# Autodesk Inventor assembly: ParticleLauncherwCollector
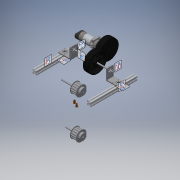
[picture p0: Inventor's stored thumbnail of the model, 180x180]
Saved by Autodesk Inventor 2016 (Build 200138000, 138)
## iProperties
Created: 2016-10-12
Part Number: ParticleLauncherwCollector
Document SubType Name: Assembly
Designer: Delta
Author: Delta
## Documents named in this file (11)
- C:\Robotics\CAD\2016-17_CAD\ParticleLauncherwCollector.iam
- C:\Robotics\CAD\COTSParts\Actobotics\555 parts\555116.ipt
- C:\Robotics\CAD\COTSParts\Actobotics\am-3102NeveRest20 (1).ipt
- C:\Robotics\CAD\COTSParts\Actobotics\634 parts\634088.ipt
- C:\Robotics\CAD\COTSParts\Wheels\4in Wheel Intergreated Hub 8mm Rev2.ipt
- C:\Robotics\CAD\COTSParts\Brecoflex\ls40t10_15-2_hub-32x10_d-8h7.ipt
- C:\Robotics\CAD\COTSParts\Actobotics\634 parts\634080.ipt
- C:\Robotics\CAD\COTSParts\Actobotics\634 parts\634078.ipt
- C:\Robotics\CAD\COTSParts\Bosch Extrusion\Bosch 20x20 9 in.ipt
- C:\Robotics\CAD\COTSParts\Actobotics\585 parts\585494.ipt
- C:\Robotics\CAD\COTSParts\Tetrix\Bronze bushing.ipt
## Components (15 placed, 10 different names)
1. 555116:1 — Insert:15
2. am-3102NeveRest20 (1):1 — Insert:15, Insert:18
3. 634088:1 — Insert:17, Insert:23, Insert:24
4. 4in Wheel Intergreated Hub 8mm Rev2:1 — Insert:17
5. 4in Wheel Intergreated Hub 8mm Rev2:2 — Insert:18
6. ls40t10_15-2_hub-32x10_d-8h7:1
7. ls40t10_15-2_hub-32x10_d-8h7:2
8. 634080:1
9. 634078:1
10. Bosch 20x20 9 in:1 — Mate:1, Flush:1, Flush:2
11. Bosch 20x20 9 in:2 — Mate:2, Flush:3
12. 585494:2 — Insert:23, Mate:1, Flush:1, Flush:2
13. 585494:3 — Insert:24, Mate:2, Flush:3
14. Bronze bushing:1
15. Bronze bushing:2
## Relationships (10: Insert 5, Flush 3, Mate 2)
- Insert:15 (-9.525 mm): 555116:1 ↔ am-3102NeveRest20 (1):1
- Insert:17 (76.2 mm): 634088:1 ↔ 4in Wheel Intergreated Hub 8mm Rev2:1
- Insert:18 (-19.05 mm): am-3102NeveRest20 (1):1 ↔ 4in Wheel Intergreated Hub 8mm Rev2:2
- Insert:23 (-12.7 mm): 634088:1 ↔ 585494:2
- Mate:1: Bosch 20x20 9 in:1 ↔ 585494:2
- Flush:1 (4.318 mm): Bosch 20x20 9 in:1 ↔ 585494:2
- Flush:2 (63.5 mm): Bosch 20x20 9 in:1 ↔ 585494:2
- Insert:24 (12.7 mm): 634088:1 ↔ 585494:3
- Mate:2: Bosch 20x20 9 in:2 ↔ 585494:3
- Flush:3 (4.318 mm): Bosch 20x20 9 in:2 ↔ 585494:3
